# Autodesk Inventor assembly: Battery and Electronics (Vertical Rack)
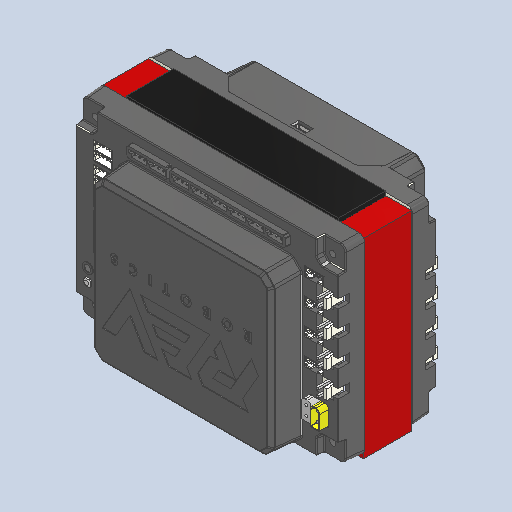
[picture p0: Inventor's stored thumbnail of the model, 512x512]
Saved by Autodesk Inventor 2022 (Build 260153000, 153)
## iProperties
Created: 2021-11-02
Part Number: Battery and Electronics (Vertical Rack)
Document SubType Name: Assembly
Designer: Admin
Author: Admin
## Documents named in this file (5)
- C:\Users\matt\Documents\Inventor\FTC\2022-23 FTC\Electronics\Battery and Electronics (Vertical Rack).iam
- C:\Users\matt\Documents\Inventor\FTC\2022-23 FTC\Electronics\Vertical Electronics Spacer.ipt
- C:\Users\matt\Documents\Inventor\FTC\2022-23 FTC\Electronics\REV-31-1153.ipt
- C:\Users\matt\Documents\Inventor\FTC\2022-23 FTC\Electronics\Battery (Approx).ipt
- C:\Users\matt\Documents\Inventor\FTC\2022-23 FTC\Fasteners\M3_S_Tapered Heat-Set Insert.ipt
## Components (8 placed, 4 different names)
1. Vertical Electronics Spacer:1 — Mate:3, Mate:9, Mate:12, Mate:13, Mate:18, Mate:19, Mate:20, Mate:21, Mate:22, Mate:23, Mate:24, Mate:25
2. REV-31-1153:2 — Mate:3, Mate:9
3. Battery (Approx):1 — Mate:12, Mate:13
4. M3_S_Tapered Heat-Set Insert:2 — Mate:21, Flush:3
5. M3_S_Tapered Heat-Set Insert:3 — Mate:22, Flush:2
6. M3_S_Tapered Heat-Set Insert:4 — Mate:20, Flush:1
7. M3_S_Tapered Heat-Set Insert:5 — Mate:18, Mate:19, Flush:1, Flush:2, Flush:3
8. REV-31-1153:3 — Mate:23, Mate:24, Mate:25
## Relationships (15: Mate 12, Flush 3)
- Mate:3: Vertical Electronics Spacer:1 ↔ REV-31-1153:2
- Mate:9: Vertical Electronics Spacer:1 ↔ REV-31-1153:2
- Mate:12: Vertical Electronics Spacer:1 ↔ Battery (Approx):1
- Mate:13: Vertical Electronics Spacer:1 ↔ Battery (Approx):1
- Mate:18: Vertical Electronics Spacer:1 ↔ M3_S_Tapered Heat-Set Insert:5
- Mate:19: Vertical Electronics Spacer:1 ↔ M3_S_Tapered Heat-Set Insert:5
- Mate:20: Vertical Electronics Spacer:1 ↔ M3_S_Tapered Heat-Set Insert:4
- Flush:1: M3_S_Tapered Heat-Set Insert:4 ↔ M3_S_Tapered Heat-Set Insert:5
- Mate:21: Vertical Electronics Spacer:1 ↔ M3_S_Tapered Heat-Set Insert:2
- Mate:22: Vertical Electronics Spacer:1 ↔ M3_S_Tapered Heat-Set Insert:3
- Flush:2: M3_S_Tapered Heat-Set Insert:3 ↔ M3_S_Tapered Heat-Set Insert:5
- Flush:3: M3_S_Tapered Heat-Set Insert:2 ↔ M3_S_Tapered Heat-Set Insert:5
- Mate:23: Vertical Electronics Spacer:1 ↔ REV-31-1153:3
- Mate:24: Vertical Electronics Spacer:1 ↔ REV-31-1153:3
- Mate:25: Vertical Electronics Spacer:1 ↔ REV-31-1153:3
